# Autodesk Inventor assembly: Assembly1
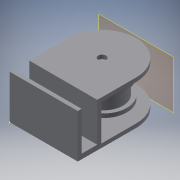
[picture p0: Inventor's stored thumbnail of the model, 180x180]
Saved by Autodesk Inventor 2016 (Build 200138000, 138)
## iProperties
Created: 2016-04-11
Part Number: Assembly1
Document SubType Name: Assembly
Designer: Thetheos
Author: Thetheos
## Documents named in this file (3)
- D:\document\3D printer\Delta Imprimante 3D\maintiens poullie\Assembly1.iam
- D:\document\3D printer\Delta Imprimante 3D\maintiens poullie\Maintients poullies V4.ipt
- D:\document\3D printer\Delta Imprimante 3D\Poulie\poulie v2.ipt
## Components (2 placed, 2 different names)
1. Maintients poullies V4:1 — Mate:1, Rotation:1
2. poulie v2:1 — Mate:1, Rotation:1
## Relationships (2: Mate 1, RelateRotation 1)
- Mate:1 (2 mm): Maintients poullies V4:1 ↔ poulie v2:1
- Rotation:1 [RelateRotation] (5 ul): Maintients poullies V4:1 ↔ poulie v2:1
